# Autodesk Inventor assembly: ASTRA
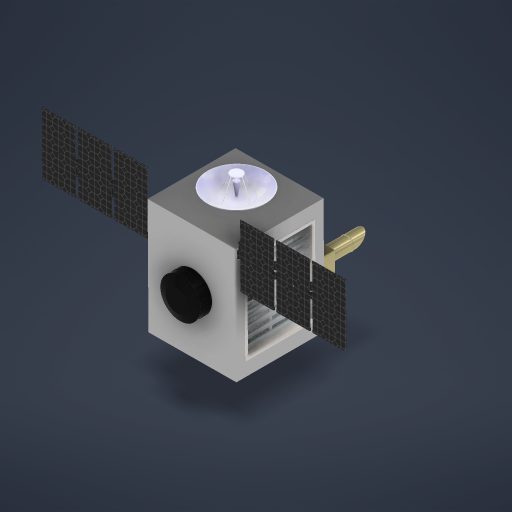
[picture p0: Inventor's stored thumbnail of the model, 512x512]
Saved by Autodesk Inventor 2023.2 (Build 272271030, 271C)
## iProperties
Created: 2023-04-10
Part Number: ASTRA
Document SubType Name: Assembly
Designer: ckeer
Author: ckeer
## Documents named in this file (10)
- D:\Github\School\Prelim\CAD\ASTRA.iam
- D:\Github\School\Prelim\CAD\ASTRA_Body.ipt
- D:\Github\School\Prelim\CAD\automatic-louver-1.snapshot.9\Zip Folder\Louver 061516\Louver 061516\Louver 061516.iam
- D:\Github\School\Prelim\CAD\Sparkwing CAD models 20220411\Sparkwing 1070x570mm 3Panel SA Deployed STEP\Sparkwing 1070x570mm 3Panel SA Deployed STEP.iam
- C:\Users\ckeer\Downloads\RIT 2X ION THRUSTER\RIT 2X ION THRUSTER.ipt
- C:\Users\ckeer\Downloads\Dish\Dish.ipt
- C:\Users\ckeer\Downloads\OTES\OTES.ipt
- D:\Github\School\Prelim\CAD\Liquid Engine.ipt
- C:\Users\ckeer\Downloads\arm assembly\arm assembly.ipt
- C:\Users\ckeer\Downloads\arm\arm.ipt
## Components (11 placed, 9 different names)
1. ASTRA_Body:1 — Mate:1, Angle:1, Mate:2, Mate:3, Mate:4, Angle:2, Mate:5, Mate:6, Mate:7, Mate:8, Mate:9, Mate:10, Mate:11, Mate:12, Mate:13, Mate:14, Mate:15, Mate:16, Mate:17, Mate:18, Mate:19
2. Louver 061516:1 [sub-assembly]
3. Louver 061516:2 [sub-assembly]
4. Sparkwing 1070x570mm 3Panel SA Deployed STEP:1 [sub-assembly] — Mate:4, Angle:2, Mate:5, Mate:6
5. Sparkwing 1070x570mm 3Panel SA Deployed STEP:2 [sub-assembly] — Mate:1, Angle:1, Mate:2, Mate:3
6. RIT 2X ION THRUSTER:1 — Mate:7, Mate:9, Mate:10
7. Dish:1 — Mate:8
8. OTES:1 — Mate:11, Mate:12, Mate:13
9. Liquid Engine:1 — Mate:14, Mate:15, Mate:16
10. arm assembly:1
11. arm:1 — Mate:17, Mate:18, Mate:19
## Relationships (21: Mate 19, Angle 2)
- Mate:1: ASTRA_Body:1 ↔ Sparkwing 1070x570mm 3Panel SA Deployed STEP:2
- Angle:1 (-90 deg): ASTRA_Body:1 ↔ Sparkwing 1070x570mm 3Panel SA Deployed STEP:2
- Mate:2 (-50.8 mm): ASTRA_Body:1 ↔ Sparkwing 1070x570mm 3Panel SA Deployed STEP:2
- Mate:3 (-635 mm): ASTRA_Body:1 ↔ Sparkwing 1070x570mm 3Panel SA Deployed STEP:2
- Mate:4: ASTRA_Body:1 ↔ Sparkwing 1070x570mm 3Panel SA Deployed STEP:1
- Angle:2 (0 deg): ASTRA_Body:1 ↔ Sparkwing 1070x570mm 3Panel SA Deployed STEP:1
- Mate:5 (-50.8 mm): ASTRA_Body:1 ↔ Sparkwing 1070x570mm 3Panel SA Deployed STEP:1
- Mate:6 (-635 mm): ASTRA_Body:1 ↔ Sparkwing 1070x570mm 3Panel SA Deployed STEP:1
- Mate:7: ASTRA_Body:1 ↔ RIT 2X ION THRUSTER:1
- Mate:8: ASTRA_Body:1 ↔ Dish:1
- Mate:9 (-750 mm): ASTRA_Body:1 ↔ RIT 2X ION THRUSTER:1
- Mate:10 (-996.95 mm): ASTRA_Body:1 ↔ RIT 2X ION THRUSTER:1
- Mate:11: ASTRA_Body:1 ↔ OTES:1
- Mate:12 (-508 mm): ASTRA_Body:1 ↔ OTES:1
- Mate:13 (-1016 mm): ASTRA_Body:1 ↔ OTES:1
- Mate:14: ASTRA_Body:1 ↔ Liquid Engine:1
- Mate:15 (-750 mm): ASTRA_Body:1 ↔ Liquid Engine:1
- Mate:16 (-750 mm): ASTRA_Body:1 ↔ Liquid Engine:1
- Mate:17: ASTRA_Body:1 ↔ arm:1
- Mate:18 (-750 mm): ASTRA_Body:1 ↔ arm:1
- Mate:19 (-508 mm): ASTRA_Body:1 ↔ arm:1
